# Autodesk Inventor assembly: 조립품1
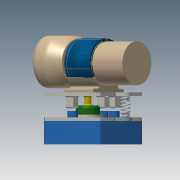
[picture p0: Inventor's stored thumbnail of the model, 180x180]
Saved by Autodesk Inventor 2015 (Build 190159000, 159)
## iProperties
Created: 2017-05-31
Part Number: 조립품1
Document SubType Name: Assembly
Designer: gatew
Author: gatew
## Documents named in this file (8)
- C:\Users\gatew\Desktop\특허\조립품1.iam
- C:\Users\gatew\Desktop\특허\arduino case.ipt
- C:\Users\gatew\Desktop\특허\bt cover.ipt
- C:\Users\gatew\Desktop\특허\cover.ipt
- C:\Users\gatew\Desktop\특허\ball joint.iam
- C:\Users\gatew\Desktop\특허\torsion spring.ipt
- C:\Users\gatew\Desktop\특허\BAND Case.ipt
- C:\Users\gatew\Desktop\특허\부품1.ipt
## Components (7 placed, 7 different names)
1. arduino case:1 — 메이트:3, 메이트:4, 메이트:5, 메이트:6, 메이트:7
2. bt cover:1 — 메이트:3, 메이트:4
3. cover:1 — 메이트:5, 메이트:6, 메이트:7, 메이트:8, 메이트:9
4. ball joint:1 [sub-assembly] — 메이트:8, 메이트:9, 메이트:10
5. torsion spring:1
6. BAND Case:1 — 메이트:10
7. 부품1:1
## Relationships (8: Mate 8)
- 메이트:3 [Mate] (0.5 mm): arduino case:1 ↔ bt cover:1
- 메이트:4 [Mate] (0.5 mm): arduino case:1 ↔ bt cover:1
- 메이트:5 [Mate]: arduino case:1 ↔ cover:1
- 메이트:6 [Mate]: arduino case:1 ↔ cover:1
- 메이트:7 [Mate]: arduino case:1 ↔ cover:1
- 메이트:8 [Mate]: cover:1 ↔ ball joint:1
- 메이트:9 [Mate]: cover:1 ↔ ball joint:1
- 메이트:10 [Mate]: ball joint:1 ↔ BAND Case:1
